# Autodesk Inventor assembly: Bevels_assem
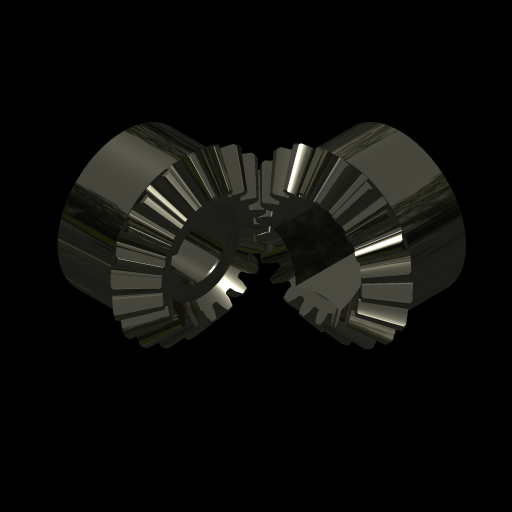
[picture p0: Inventor's stored thumbnail of the model, 512x512]
Saved by Autodesk Inventor 2023 (Build 270158030, 158C)
## iProperties
Created: 2022-10-27
Part Number: Bevels_assem
Document SubType Name: Assembly
Designer: kumpu
Author: kumpu
## Documents named in this file (3)
- C:\Users\kumpu\Documents\SBU\CAD\SBRT\Robocup Rescue\Drive\v1\Bevels_assem.iam
- C:\Users\kumpu\Documents\SBU\CAD\SBSR\REV 06\am-3772 1.25, 20T, 500 Hex Bore.ipt
- C:\Users\kumpu\Documents\SBU\CAD\SBSR\REV 06\am-3776 Miter Gear 1.25, 20T, 8mm, 2mm Key Bore.ipt
## Components (2 placed, 2 different names)
1. am-3772 1.25, 20T, 500 Hex Bore:1 — Mate:1, Mate:2, Mate:4
2. am-3776 Miter Gear 1.25, 20T, 8mm, 2mm Key Bore:1 — Mate:3, Mate:5
## Relationships (5: Mate 5)
- Mate:1: am-3772 1.25, 20T, 500 Hex Bore:1
- Mate:2: am-3772 1.25, 20T, 500 Hex Bore:1
- Mate:3: am-3776 Miter Gear 1.25, 20T, 8mm, 2mm Key Bore:1
- Mate:4 (-23.114 mm): am-3772 1.25, 20T, 500 Hex Bore:1
- Mate:5 (-23.114 mm): am-3776 Miter Gear 1.25, 20T, 8mm, 2mm Key Bore:1
